# Autodesk Inventor assembly: Hexapod
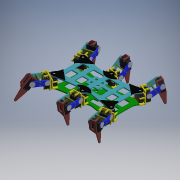
[picture p0: Inventor's stored thumbnail of the model, 180x180]
Saved by Autodesk Inventor 2017 (Build 210142000, 142)
## iProperties
Part Number: Hexapod
Document SubType Name: Assembly
Designer: Alexander Miller
Author: Alexander Miller
## Documents named in this file (10)
- D:\Alexander Miller\Documents\Git\Hexapod\3DParts\Hexapod.iam
- D:\Alexander Miller\Documents\Git\Hexapod\3DParts\Body_bottom.ipt
- D:\Alexander Miller\Documents\Git\Hexapod\3DParts\leg_right.iam
- D:\Alexander Miller\Documents\Git\Hexapod\3DParts\Body_top.ipt
- D:\Alexander Miller\Documents\Git\Hexapod\3DParts\Servo.ipt
- D:\Alexander Miller\Documents\Git\Hexapod\3DParts\Servo_arm.ipt
- D:\Alexander Miller\Documents\Git\Hexapod\3DParts\ball_bearing.ipt
- D:\Alexander Miller\Documents\Git\Hexapod\3DParts\leg_left.iam
- D:\Alexander Miller\Documents\Git\Hexapod\3DParts\Connector.ipt
- D:\Alexander Miller\Documents\Git\Hexapod\3DParts\Body_top_extras.ipt
## Components (21 placed, 7 different names)
1. leg_right:1 [sub-assembly] — Rigid:16, Rigid:22
2. leg_right:2 [sub-assembly] — Rigid:17, Rigid:26
3. leg_right:3 [sub-assembly] — Rigid:18, Rigid:27
4. Body_top:1 — Rigid:22, Rigid:23, Rigid:24, Rigid:25, Rigid:27, Rigid:26, Rigid:28
5. Body_bottom:1 — Rigid:7, Rigid:8, Rigid:9, Rigid:10, Rigid:11, Rigid:12
6. ball_bearing:1 — Rigid:7, Rotational:1
7. ball_bearing:2 — Rigid:12, Rotational:4
8. ball_bearing:3 — Rigid:11, Rotational:5
9. ball_bearing:4 — Rigid:8, Rotational:2
10. ball_bearing:5 — Rigid:10, Rotational:3
11. ball_bearing:6 — Rigid:9, Rotational:6
12. leg_left:1 [sub-assembly] — Rigid:19, Rigid:23
13. leg_left:2 [sub-assembly] — Rigid:20, Rigid:24
14. leg_left:3 [sub-assembly] — Rigid:21, Rigid:25
15. Connector:1 — Rigid:16, Rotational:1
16. Connector:2 — Rigid:17, Rotational:6
17. Connector:3 — Rigid:18, Rotational:5
18. Connector:4 — Rigid:19, Rotational:2
19. Connector:5 — Rigid:20, Rotational:3
20. Connector:6 — Rigid:21, Rotational:4
21. Body_top_extras:1 — Rigid:28
## Relationships (25: WeldJoint 19, RevoluteJoint 6)
- Rigid:7 [WeldJoint]: Body_bottom:1 ↔ ball_bearing:1
- Rigid:8 [WeldJoint]: Body_bottom:1 ↔ ball_bearing:4
- Rigid:9 [WeldJoint]: Body_bottom:1 ↔ ball_bearing:6
- Rigid:10 [WeldJoint]: Body_bottom:1 ↔ ball_bearing:5
- Rigid:11 [WeldJoint]: Body_bottom:1 ↔ ball_bearing:3
- Rigid:12 [WeldJoint]: Body_bottom:1 ↔ ball_bearing:2
- Rigid:16 [WeldJoint]: leg_right:1 ↔ Connector:1
- Rigid:17 [WeldJoint]: leg_right:2 ↔ Connector:2
- Rigid:18 [WeldJoint]: leg_right:3 ↔ Connector:3
- Rigid:19 [WeldJoint]: leg_left:1 ↔ Connector:4
- Rigid:20 [WeldJoint]: leg_left:2 ↔ Connector:5
- Rigid:21 [WeldJoint]: leg_left:3 ↔ Connector:6
- Rigid:22 [WeldJoint]: leg_right:1 ↔ Body_top:1
- Rigid:23 [WeldJoint]: Body_top:1 ↔ leg_left:1
- Rigid:24 [WeldJoint]: Body_top:1 ↔ leg_left:2
- Rigid:25 [WeldJoint]: Body_top:1 ↔ leg_left:3
- Rigid:27 [WeldJoint]: leg_right:3 ↔ Body_top:1
- Rigid:26 [WeldJoint]: leg_right:2 ↔ Body_top:1
- Rotational:1 [RevoluteJoint]: ball_bearing:1 ↔ Connector:1
- Rotational:2 [RevoluteJoint]: ball_bearing:4 ↔ Connector:4
- Rotational:3 [RevoluteJoint]: ball_bearing:5 ↔ Connector:5
- Rotational:4 [RevoluteJoint]: ball_bearing:2 ↔ Connector:6
- Rotational:5 [RevoluteJoint]: ball_bearing:3 ↔ Connector:3
- Rotational:6 [RevoluteJoint]: ball_bearing:6 ↔ Connector:2
- Rigid:28 [WeldJoint]: Body_top:1 ↔ Body_top_extras:1
## Named parameters: b_mat_thickness = 5 mm, s_height = 38 mm, s_shaft_height = 6 mm, sa_thickness = 2 mm
